# Autodesk Inventor assembly: spool
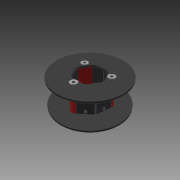
[picture p0: Inventor's stored thumbnail of the model, 180x180]
Saved by Autodesk Inventor 2014 (Build 180170000, 170)
## iProperties
Created: 2014-04-05
Part Number: spool
Document SubType Name: Assembly
Designer: buben
Author: buben
## Documents named in this file (11)
- C:\Users\buben\Documents\GitHub\bspool\inventor_files\assemblies\spool.iam
- C:\Users\buben\Documents\GitHub\bspool\inventor_files\parts\spool_a.ipt
- C:\Users\buben\Documents\GitHub\bspool\inventor_files\parts\spool_brace.ipt
- C:\Users\buben\Documents\GitHub\bspool\inventor_files\parts\spool_b.ipt
- C:\Users\buben\Documents\Inventor\Content Center Files\R2014\en-US\CSN 02 1702  B\CSN 02 1702 - B 4,3.ipt
- C:\Users\buben\Documents\Inventor\Content Center Files\R2014\en-US\ISO 4762(2)\ISO 4762 - M4 x 20ISO.ipt
- C:\Users\buben\Documents\Inventor\Content Center Files\R2014\en-US\ISO 7040\ISO 7040 - M4.ipt
- C:\Users\buben\Documents\GitHub\bspool\inventor_files\parts\filament_guide.ipt
- C:\Users\buben\Documents\GitHub\bspool\inventor_files\utils\washer_m8_wood.ipt
- C:\Users\buben\Documents\Inventor\Content Center Files\R2014\en-US\DIN 931-1\DIN 931-1 - M8 x 80.ipt
- C:\Users\buben\Documents\GitHub\bspool\inventor_files\parts\spool_hex_holder.ipt
## Components (47 placed, 10 different names)
1. spool_a:1 — Mate:1, Mate:2, Mate:3, Mate:4, Mate:5, Mate:6, Mate:7, Mate:8, Mate:9, Mate:10, Mate:11, Mate:12, Mate:13, Mate:14, Mate:15, Mate:16, Mate:17, Mate:18, Mate:19, Mate:20, Mate:21, Mate:23, Mate:24, Mate:25, Mate:26, Mate:27, Mate:28, Mate:29, Mate:30, Mate:31, Mate:32, Mate:33, Mate:34, Mate:35, Mate:36, Mate:61, Mate:62, Mate:63, Mate:70, Mate:71, Mate:72, Mate:73, Mate:74, Mate:75, Angle:1, Angle:2, Angle:3
2. spool_brace:1 — Mate:5, Mate:20, Mate:21, Mate:45, Mate:66
3. spool_brace:2 — Mate:4, Mate:18, Mate:19, Mate:22, Mate:43, Mate:69
4. spool_brace:3 — Mate:6, Mate:16, Mate:17, Mate:41, Mate:68
5. spool_brace:4 — Mate:7, Mate:14, Mate:15, Mate:39, Mate:65
6. spool_brace:5 — Mate:8, Mate:12, Mate:13, Mate:37, Mate:64
7. spool_brace:6 — Mate:9, Mate:10, Mate:11, Mate:47, Mate:67
8. spool_b:1 — Mate:22, Mate:23, Mate:24, Mate:76, Mate:77, Mate:78, Mate:79, Mate:80, Mate:81
9. CSN 02 1702 B B 4,3:1 — Mate:47, Mate:48, Mate:59
10. CSN 02 1702 B B 4,3:2 — Mate:43, Mate:44, Mate:55
11. CSN 02 1702 B B 4,3:3 — Mate:37, Mate:38, Mate:49
12. CSN 02 1702 B B 4,3:4 — Mate:45, Mate:46, Mate:57
13. CSN 02 1702 B B 4,3:5 — Mate:35, Mate:36, Insert:5
14. CSN 02 1702 B B 4,3:6 — Mate:33, Mate:34, Insert:3
15. CSN 02 1702 B B 4,3:7 — Mate:41, Mate:42, Mate:53
16. CSN 02 1702 B B 4,3:8 — Mate:39, Mate:40, Mate:51
17. CSN 02 1702 B B 4,3:9 — Mate:29, Mate:30, Insert:6
18. CSN 02 1702 B B 4,3:10 — Mate:31, Mate:32, Insert:1
19. CSN 02 1702 B B 4,3:11 — Mate:27, Mate:28, Insert:4
20. CSN 02 1702 B B 4,3:12 — Mate:25, Mate:26, Insert:2
21. ISO 4762 M4 x 20:1 — Insert:1, Mate:46, Mate:58
22. ISO 4762 M4 x 20:2 — Insert:2, Mate:48, Mate:60
23. ISO 4762 M4 x 20:3 — Insert:3, Mate:44, Mate:56
24. ISO 4762 M4 x 20:4 — Insert:4, Mate:38, Mate:50
25. ISO 4762 M4 x 20:5 — Insert:5, Mate:42, Mate:54
26. ISO 4762 M4 x 20:6 — Insert:6, Mate:40, Mate:52
27. DIN EN ISO 7040 M4:1 — Mate:53, Mate:54
28. DIN EN ISO 7040 M4:2 — Mate:57, Mate:58
29. DIN EN ISO 7040 M4:3 — Mate:59, Mate:60
30. DIN EN ISO 7040 M4:4 — Mate:51, Mate:52
31. DIN EN ISO 7040 M4:5 — Mate:49, Mate:50
32. DIN EN ISO 7040 M4:6 — Mate:55, Mate:56
33. filament_guide:1 — Mate:62, Mate:64, Mate:65
34. filament_guide:2 — Mate:61, Mate:68, Mate:69
35. filament_guide:3 — Mate:63, Mate:66, Mate:67
36. washer_m8_wood:1 — Mate:70, Mate:71, Insert:8, Mate:82
37. washer_m8_wood:2 — Mate:74, Mate:75, Insert:9, Mate:83
38. washer_m8_wood:3 — Mate:72, Mate:73, Insert:7, Mate:84
39. washer_m8_wood:4 — Mate:76, Mate:77
40. washer_m8_wood:5 — Mate:78, Mate:79
41. washer_m8_wood:6 — Mate:80, Mate:81
42. DIN 931-1 - replaced by DIN EN 24014 M8 x 80:1 — Insert:9, Mate:87, Mate:88
43. DIN 931-1 - replaced by DIN EN 24014 M8 x 80:2 — Insert:8, Mate:85, Mate:86
44. DIN 931-1 - replaced by DIN EN 24014 M8 x 80:3 — Insert:7, Mate:89, Mate:90
45. spool_hex_holder:1 — Mate:82, Mate:85, Mate:86, Angle:1
46. spool_hex_holder:2 — Mate:84, Mate:89, Mate:90, Angle:3
47. spool_hex_holder:3 — Mate:83, Mate:87, Mate:88, Angle:2
## Relationships (102: Mate 90, Insert 9, Angle 3)
- Mate:1: spool_a:1
- Mate:2: spool_a:1
- Mate:3: spool_a:1
- Mate:4: spool_a:1 ↔ spool_brace:2
- Mate:5: spool_a:1 ↔ spool_brace:1
- Mate:6: spool_a:1 ↔ spool_brace:3
- Mate:7: spool_a:1 ↔ spool_brace:4
- Mate:8: spool_a:1 ↔ spool_brace:5
- Mate:9: spool_a:1 ↔ spool_brace:6
- Mate:10: spool_a:1 ↔ spool_brace:6
- Mate:11: spool_a:1 ↔ spool_brace:6
- Mate:12: spool_a:1 ↔ spool_brace:5
- Mate:13: spool_a:1 ↔ spool_brace:5
- Mate:14: spool_a:1 ↔ spool_brace:4
- Mate:15: spool_a:1 ↔ spool_brace:4
- Mate:16: spool_a:1 ↔ spool_brace:3
- Mate:17: spool_a:1 ↔ spool_brace:3
- Mate:18: spool_a:1 ↔ spool_brace:2
- Mate:19: spool_a:1 ↔ spool_brace:2
- Mate:20: spool_a:1 ↔ spool_brace:1
- Mate:21: spool_a:1 ↔ spool_brace:1
- Mate:22: spool_brace:2 ↔ spool_b:1
- Mate:23: spool_a:1 ↔ spool_b:1
- Mate:24: spool_a:1 ↔ spool_b:1
- Mate:25: spool_a:1 ↔ CSN 02 1702 B B 4,3:12
- Mate:26: spool_a:1 ↔ CSN 02 1702 B B 4,3:12
- Mate:27: spool_a:1 ↔ CSN 02 1702 B B 4,3:11
- Mate:28: spool_a:1 ↔ CSN 02 1702 B B 4,3:11
- Mate:29: spool_a:1 ↔ CSN 02 1702 B B 4,3:9
- Mate:30: spool_a:1 ↔ CSN 02 1702 B B 4,3:9
- Mate:31: spool_a:1 ↔ CSN 02 1702 B B 4,3:10
- Mate:32: spool_a:1 ↔ CSN 02 1702 B B 4,3:10
- Mate:33: spool_a:1 ↔ CSN 02 1702 B B 4,3:6
- Mate:34: spool_a:1 ↔ CSN 02 1702 B B 4,3:6
- Mate:35: spool_a:1 ↔ CSN 02 1702 B B 4,3:5
- Mate:36: spool_a:1 ↔ CSN 02 1702 B B 4,3:5
- Insert:1: CSN 02 1702 B B 4,3:10 ↔ ISO 4762 M4 x 20:1
- Insert:2: CSN 02 1702 B B 4,3:12 ↔ ISO 4762 M4 x 20:2
- Insert:3: CSN 02 1702 B B 4,3:6 ↔ ISO 4762 M4 x 20:3
- Insert:4: CSN 02 1702 B B 4,3:11 ↔ ISO 4762 M4 x 20:4
- Insert:5: CSN 02 1702 B B 4,3:5 ↔ ISO 4762 M4 x 20:5
- Insert:6: CSN 02 1702 B B 4,3:9 ↔ ISO 4762 M4 x 20:6
- Mate:37: spool_brace:5 ↔ CSN 02 1702 B B 4,3:3
- Mate:38: CSN 02 1702 B B 4,3:3 ↔ ISO 4762 M4 x 20:4
- Mate:39: spool_brace:4 ↔ CSN 02 1702 B B 4,3:8
- Mate:40: CSN 02 1702 B B 4,3:8 ↔ ISO 4762 M4 x 20:6
- Mate:41: spool_brace:3 ↔ CSN 02 1702 B B 4,3:7
- Mate:42: CSN 02 1702 B B 4,3:7 ↔ ISO 4762 M4 x 20:5
- Mate:43: spool_brace:2 ↔ CSN 02 1702 B B 4,3:2
- Mate:44: CSN 02 1702 B B 4,3:2 ↔ ISO 4762 M4 x 20:3
- Mate:45: spool_brace:1 ↔ CSN 02 1702 B B 4,3:4
- Mate:46: CSN 02 1702 B B 4,3:4 ↔ ISO 4762 M4 x 20:1
- Mate:47: spool_brace:6 ↔ CSN 02 1702 B B 4,3:1
- Mate:48: CSN 02 1702 B B 4,3:1 ↔ ISO 4762 M4 x 20:2
- Mate:49: CSN 02 1702 B B 4,3:3 ↔ DIN EN ISO 7040 M4:5
- Mate:50: ISO 4762 M4 x 20:4 ↔ DIN EN ISO 7040 M4:5
- Mate:51: CSN 02 1702 B B 4,3:8 ↔ DIN EN ISO 7040 M4:4
- Mate:52: ISO 4762 M4 x 20:6 ↔ DIN EN ISO 7040 M4:4
- Mate:53: CSN 02 1702 B B 4,3:7 ↔ DIN EN ISO 7040 M4:1
- Mate:54: ISO 4762 M4 x 20:5 ↔ DIN EN ISO 7040 M4:1
- Mate:55: CSN 02 1702 B B 4,3:2 ↔ DIN EN ISO 7040 M4:6
- Mate:56: ISO 4762 M4 x 20:3 ↔ DIN EN ISO 7040 M4:6
- Mate:57: CSN 02 1702 B B 4,3:4 ↔ DIN EN ISO 7040 M4:2
- Mate:58: ISO 4762 M4 x 20:1 ↔ DIN EN ISO 7040 M4:2
- Mate:59: CSN 02 1702 B B 4,3:1 ↔ DIN EN ISO 7040 M4:3
- Mate:60: ISO 4762 M4 x 20:2 ↔ DIN EN ISO 7040 M4:3
- Mate:61: spool_a:1 ↔ filament_guide:2
- Mate:62: spool_a:1 ↔ filament_guide:1
- Mate:63: spool_a:1 ↔ filament_guide:3
- Mate:64: spool_brace:5 ↔ filament_guide:1
- Mate:65: spool_brace:4 ↔ filament_guide:1
- Mate:66: spool_brace:1 ↔ filament_guide:3
- Mate:67: spool_brace:6 ↔ filament_guide:3
- Mate:68: spool_brace:3 ↔ filament_guide:2
- Mate:69: spool_brace:2 ↔ filament_guide:2
- Mate:70: spool_a:1 ↔ washer_m8_wood:1
- Mate:71: spool_a:1 ↔ washer_m8_wood:1
- Mate:72: spool_a:1 ↔ washer_m8_wood:3
- Mate:73: spool_a:1 ↔ washer_m8_wood:3
- Mate:74: spool_a:1 ↔ washer_m8_wood:2
- Mate:75: spool_a:1 ↔ washer_m8_wood:2
- Mate:76: spool_b:1 ↔ washer_m8_wood:4
- Mate:77: spool_b:1 ↔ washer_m8_wood:4
- Mate:78: spool_b:1 ↔ washer_m8_wood:5
- Mate:79: spool_b:1 ↔ washer_m8_wood:5
- Mate:80: spool_b:1 ↔ washer_m8_wood:6
- Mate:81: spool_b:1 ↔ washer_m8_wood:6
- Insert:7: washer_m8_wood:3 ↔ DIN 931-1 - replaced by DIN EN 24014 M8 x 80:3
- Insert:8: washer_m8_wood:1 ↔ DIN 931-1 - replaced by DIN EN 24014 M8 x 80:2
- Insert:9: washer_m8_wood:2 ↔ DIN 931-1 - replaced by DIN EN 24014 M8 x 80:1
- Mate:82: washer_m8_wood:1 ↔ spool_hex_holder:1
- Mate:83: washer_m8_wood:2 ↔ spool_hex_holder:3
- Mate:84: washer_m8_wood:3 ↔ spool_hex_holder:2
- Mate:85: DIN 931-1 - replaced by DIN EN 24014 M8 x 80:2 ↔ spool_hex_holder:1
- Mate:86: DIN 931-1 - replaced by DIN EN 24014 M8 x 80:2 ↔ spool_hex_holder:1
- Mate:87: DIN 931-1 - replaced by DIN EN 24014 M8 x 80:1 ↔ spool_hex_holder:3
- Mate:88: DIN 931-1 - replaced by DIN EN 24014 M8 x 80:1 ↔ spool_hex_holder:3
- Mate:89: DIN 931-1 - replaced by DIN EN 24014 M8 x 80:3 ↔ spool_hex_holder:2
- Mate:90: DIN 931-1 - replaced by DIN EN 24014 M8 x 80:3 ↔ spool_hex_holder:2
- Angle:1 (0 deg): spool_a:1 ↔ spool_hex_holder:1
- Angle:2 (0 deg): spool_a:1 ↔ spool_hex_holder:3
- Angle:3 (0 deg): spool_a:1 ↔ spool_hex_holder:2
